# Autodesk Inventor assembly: Rover
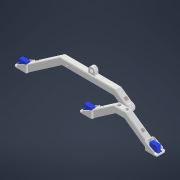
[picture p0: Inventor's stored thumbnail of the model, 180x180]
Saved by Autodesk Inventor 2021 (Build 250183000, 183)
## iProperties
Created: 2021-01-03
Part Number: Rover
Document SubType Name: Assembly
Designer: laure
Author: laure
## Documents named in this file (6)
- E:\Projects\Rover\Rover.iam
- E:\Projects\Rover\Rocker_hinten.ipt
- E:\Projects\Rover\Rocker_vorne.ipt
- E:\Projects\Rover\Servohalterung.ipt
- E:\Projects\Rover\Bogie.ipt
- E:\Projects\Rover\MicroServo.ipt
## Components (9 placed, 5 different names)
1. Fahrwerk_rocker_hinten:1 — Passend:3, Passend:4, Drehbar:1
2. Fahrwerk_rocker_vorne:1 — Passend:1, Passend:2, Passend:3, Passend:4
3. Servohalterung:1 — Passend:1, Passend:2, Passend:9, Passend:10
4. Servohalterung:2 — Passend:5, Passend:6, Passend:11, Passend:12
5. Servohalterung:3 — Passend:7, Passend:8, Passend:13, Passend:14
6. Fahrwerk_bogie:1 — Passend:5, Passend:6, Passend:7, Passend:8, Drehbar:1
7. MicroServo:1 — Passend:9, Passend:10
8. MicroServo:2 — Passend:11, Passend:12
9. MicroServo:3 — Passend:13, Passend:14
## Relationships (15: Mate 14, RevoluteJoint 1)
- Passend:1 [Mate]: Fahrwerk_rocker_vorne:1 ↔ Servohalterung:1
- Passend:2 [Mate]: Fahrwerk_rocker_vorne:1 ↔ Servohalterung:1
- Passend:3 [Mate]: Fahrwerk_rocker_hinten:1 ↔ Fahrwerk_rocker_vorne:1
- Passend:4 [Mate]: Fahrwerk_rocker_hinten:1 ↔ Fahrwerk_rocker_vorne:1
- Passend:5 [Mate]: Servohalterung:2 ↔ Fahrwerk_bogie:1
- Passend:6 [Mate]: Servohalterung:2 ↔ Fahrwerk_bogie:1
- Passend:7 [Mate]: Servohalterung:3 ↔ Fahrwerk_bogie:1
- Passend:8 [Mate]: Servohalterung:3 ↔ Fahrwerk_bogie:1
- Drehbar:1 [RevoluteJoint]: Fahrwerk_rocker_hinten:1 ↔ Fahrwerk_bogie:1
- Passend:9 [Mate]: Servohalterung:1 ↔ MicroServo:1
- Passend:10 [Mate]: Servohalterung:1 ↔ MicroServo:1
- Passend:11 [Mate]: Servohalterung:2 ↔ MicroServo:2
- Passend:12 [Mate]: Servohalterung:2 ↔ MicroServo:2
- Passend:13 [Mate]: Servohalterung:3 ↔ MicroServo:3
- Passend:14 [Mate]: Servohalterung:3 ↔ MicroServo:3
